# Autodesk Inventor assembly: belt_clip_assembly
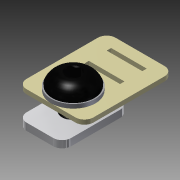
[picture p0: Inventor's stored thumbnail of the model, 180x180]
Saved by Autodesk Inventor 2014 (Build 180170000, 170)
## iProperties
Created: 2013-05-31
Part Number: belt_clip_assembly
Document SubType Name: Assembly
Designer: Edward
Mass: 2.88191 g
Surface Area: 15.4013 cm^2
Volume: 0.765461 cm^3
Density: 3.76494 g/cm^3
Author: Edward
## Documents named in this file (5)
- C:\Users\Edward\Documents\Vault\Designs\Shapeoko_v2\v2_final\belt_clip_assembly.iam
- C:\Users\Edward\Documents\Vault\Designs\Shapeoko_v2\v2_final\belt_clip.ipt
- C:\Users\Edward\Documents\Vault\Designs\Shapeoko_v2\v2_final\91239A222.ipt
- C:\Users\Edward\Documents\Vault\Designs\Shapeoko_v2\v2_final\25287-02.ipt
- C:\Users\Edward\Documents\Vault\Designs\Shapeoko_v2\v2_final\26016-01.ipt
## Components (4 placed, 4 different names)
1. belt_clip:1 — Insert:2, Insert:3, Angle:1
2. 91239A222:1 — Insert:1
3. 25287-02:1 — Insert:1, Insert:2
4. 26016-01:1 — Insert:3, Angle:1
## Relationships (4: Insert 3, Angle 1)
- Insert:1: 91239A222:1 ↔ 25287-02:1
- Insert:2: belt_clip:1 ↔ 25287-02:1
- Insert:3 (3 mm): belt_clip:1 ↔ 26016-01:1
- Angle:1 (0 deg): belt_clip:1 ↔ 26016-01:1
